# Autodesk Inventor assembly: S-GH-304-CM
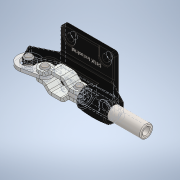
[picture p0: Inventor's stored thumbnail of the model, 180x180]
Saved by Autodesk Inventor 2021 (Build 250183000, 183)
## iProperties
Created: 2019-11-12
Part Number: S-GH-304-CM
Description: STEP AP214
Document SubType Name: Assembly
Designer: nelso
Sending System: SolidWorks 2018
Preprocessor: SwSTEP 2.0
Title: S-GH-304-CM.STEP
Revision Number: ANY
## Documents named in this file (6)
- C:\Users\nelso\Desktop\Soporte paciente espinografia\Soporte Paciente Espinografia\Workspaces\Workspace\S-GH-304-CM.iam
- C:\Users\nelso\Desktop\Soporte paciente espinografia\Soporte Paciente Espinografia\Workspaces\Workspace\Cuerpo GH-304-305-CM.ipt
- C:\Users\nelso\Desktop\Soporte paciente espinografia\Soporte Paciente Espinografia\Workspaces\Workspace\Vastago GH-304-305-CM.ipt
- C:\Users\nelso\Desktop\Soporte paciente espinografia\Soporte Paciente Espinografia\Workspaces\Workspace\Viela GH-304-305-CM.ipt
- C:\Users\nelso\Desktop\Soporte paciente espinografia\Soporte Paciente Espinografia\Workspaces\Workspace\Remache 1.ipt
- C:\Users\nelso\Desktop\Soporte paciente espinografia\Soporte Paciente Espinografia\Workspaces\Workspace\palanca2.ipt
## Components (8 placed, 8 different names)
1. Cuerpo GH-304-305-CM_1 — Mate:1, Mate:13, Mate:14
2. Vastago GH-304-305-CM_2 — Mate:1, Mate:2, Mate:5, Mate:7
3. Viela GH-304-305-CM_3 — Mate:4, Mate:7, Mate:9
4. Viela GH-304-305-CM_4 — Mate:3, Mate:5, Mate:6, Mate:8, Mate:10
5. Remache 1_5 — Mate:8, Mate:9, Mate:10, Mate:15
6. Remache 1_6 — Mate:2, Mate:3, Mate:4, Mate:6
7. Remache 1_7 — Mate:13, Mate:14, Mate:17
8. palanca2:1 — Mate:15, Mate:17
## Relationships (14: Mate 14)
- Mate:1: Cuerpo GH-304-305-CM_1 ↔ Vastago GH-304-305-CM_2
- Mate:2: Vastago GH-304-305-CM_2 ↔ Remache 1_6
- Mate:3: Viela GH-304-305-CM_4 ↔ Remache 1_6
- Mate:4: Viela GH-304-305-CM_3 ↔ Remache 1_6
- Mate:5: Vastago GH-304-305-CM_2 ↔ Viela GH-304-305-CM_4
- Mate:6: Viela GH-304-305-CM_4 ↔ Remache 1_6
- Mate:7: Vastago GH-304-305-CM_2 ↔ Viela GH-304-305-CM_3
- Mate:8: Viela GH-304-305-CM_4 ↔ Remache 1_5
- Mate:9: Viela GH-304-305-CM_3 ↔ Remache 1_5
- Mate:10: Viela GH-304-305-CM_4 ↔ Remache 1_5
- Mate:13: Cuerpo GH-304-305-CM_1 ↔ Remache 1_7
- Mate:14: Cuerpo GH-304-305-CM_1 ↔ Remache 1_7
- Mate:15: Remache 1_5 ↔ palanca2:1
- Mate:17: Remache 1_7 ↔ palanca2:1
